# Autodesk Inventor assembly: WithAdapter2Inch
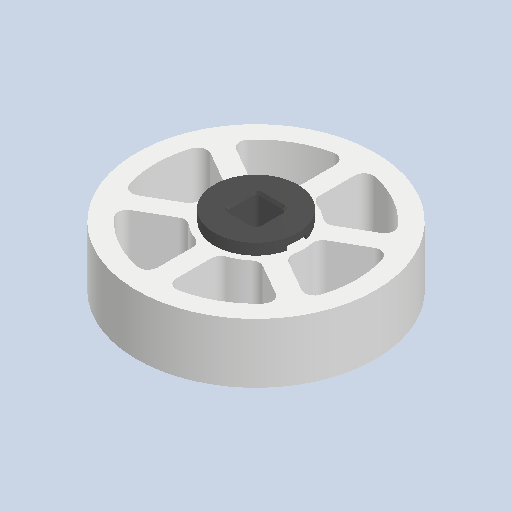
[picture p0: Inventor's stored thumbnail of the model, 512x512]
Saved by Autodesk Inventor 2023 (Build 270158000, 158)
## iProperties
Created: 2022-09-02
Part Number: WithAdapter2Inch
Document SubType Name: Assembly
Designer: alex
Author: alex
## Documents named in this file (4)
- C:\Users\alex\Documents\GitHub\4067X_spin_up_cad\WithAdapter2Inch.iam
- C:\Users\alex\Documents\GitHub\4067X_spin_up_cad\Library\Motion\Wheels\Flex Wheels\2.000 Flex Wheel\2.000 30A .500.ipt
- C:\Users\alex\Documents\GitHub\4067X_spin_up_cad\Library\Motion\Wheels\Flex Wheels\2.000 Flex Wheel.ipt
- C:\Users\alex\Documents\GitHub\4067X_spin_up_cad\Library\Motion\Wheels\Flex Wheels\VersaHex Adapters .250.ipt
## Components (3 placed, 2 different names)
1. 2.000 30A .500:1 — Mate:1, Mate:2, Mate:3, Mate:4
2. VersaHex Adapters .250:1 — Mate:1, Mate:2, Flush:1, Flush:2, Mate:4
3. VersaHex Adapters .250:2 — Flush:1, Flush:2, Mate:3
## Relationships (6: Mate 4, Flush 2)
- Mate:1 (-1.6002 mm): 2.000 30A .500:1 ↔ VersaHex Adapters .250:1
- Mate:2 (-1.6002 mm): 2.000 30A .500:1 ↔ VersaHex Adapters .250:1
- Flush:1: VersaHex Adapters .250:1 ↔ VersaHex Adapters .250:2
- Flush:2: VersaHex Adapters .250:1 ↔ VersaHex Adapters .250:2
- Mate:3: 2.000 30A .500:1 ↔ VersaHex Adapters .250:2
- Mate:4: 2.000 30A .500:1 ↔ VersaHex Adapters .250:1
